# Autodesk Inventor assembly: Cuvette-rack
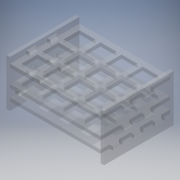
[picture p0: Inventor's stored thumbnail of the model, 180x180]
Saved by Autodesk Inventor 2018 (Build 220112000, 112)
## iProperties
Created: 2017-10-30
Part Number: Cuvette-rack
Document SubType Name: Assembly
Designer: xl0
Author: xl0
## Documents named in this file (4)
- E:\Alex\koi\Cuvette-rack\Cuvette-rack.iam
- E:\Alex\koi\Cuvette-rack\Top.ipt
- E:\Alex\koi\Cuvette-rack\Side.ipt
- E:\Alex\koi\Cuvette-rack\Bottom.ipt
## Components (5 placed, 3 different names)
1. Top:1 — Flush:1, Flush:2, Flush:3, Flush:4, Flush:5, Mate:2
2. Top:2 — Flush:4, Flush:5, Flush:6, Mate:3
3. Bottom:1 — Flush:7, Mate:1
4. Side:1 — Flush:1
5. Side:2 — Mate:1, Mate:2, Mate:3
## Relationships (10: Flush 7, Mate 3)
- Flush:1: Top:1 ↔ Side:1
- Flush:2 (15 mm): Top:1
- Flush:3 (25 mm): Top:1
- Flush:4: Top:1 ↔ Top:2
- Flush:5: Top:1 ↔ Top:2
- Flush:6: Top:2
- Flush:7: Bottom:1
- Mate:1: Bottom:1 ↔ Side:2
- Mate:2: Top:1 ↔ Side:2
- Mate:3: Top:2 ↔ Side:2
